# Autodesk Inventor assembly: Assembly1
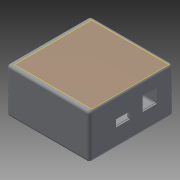
[picture p0: Inventor's stored thumbnail of the model, 180x180]
Saved by Autodesk Inventor 2013 (Build 170138000, 138)
## iProperties
Created: 2013-01-09
Part Number: Assembly1
Document SubType Name: Assembly
Designer: md
Author: md
## Documents named in this file (4)
- X:\PROJECTS\HEXASENSE\ENCLOSURE\Assembly1.iam
- X:\PROJECTS\HEXASENSE\ENCLOSURE\Unterschale.ipt
- X:\PROJECTS\HEXASENSE\ENCLOSURE\Oberschale.ipt
- C:\Users\md\Documents\Inventor\Content Center Files\R2013\en-US\ISO 7049 - C-Z(2)\ISO 7049 - ST 3,5 x 25 - C - Z.ipt
## Components (4 placed, 3 different names)
1. Unterschale:1 — Mate:5, Mate:6, Mate:7, Mate:8, Mate:9, Mate:10, Mate:11
2. Oberschale:1 — Mate:5, Mate:6, Mate:7
3. ISO 7049 - C-Z ST 3,5 x 25 - C - Z:1 — Mate:8, Mate:9
4. ISO 7049 - C-Z ST 3,5 x 25 - C - Z:2 — Mate:10, Mate:11
## Relationships (7: Mate 7)
- Mate:5: Unterschale:1 ↔ Oberschale:1
- Mate:6: Unterschale:1 ↔ Oberschale:1
- Mate:7: Unterschale:1 ↔ Oberschale:1
- Mate:9: Unterschale:1 ↔ ISO 7049 - C-Z ST 3,5 x 25 - C - Z:1
- Mate:11: Unterschale:1 ↔ ISO 7049 - C-Z ST 3,5 x 25 - C - Z:2
- Mate:8: Unterschale:1 ↔ ISO 7049 - C-Z ST 3,5 x 25 - C - Z:1
- Mate:10: Unterschale:1 ↔ ISO 7049 - C-Z ST 3,5 x 25 - C - Z:2
